# Autodesk Inventor assembly: Assembly1
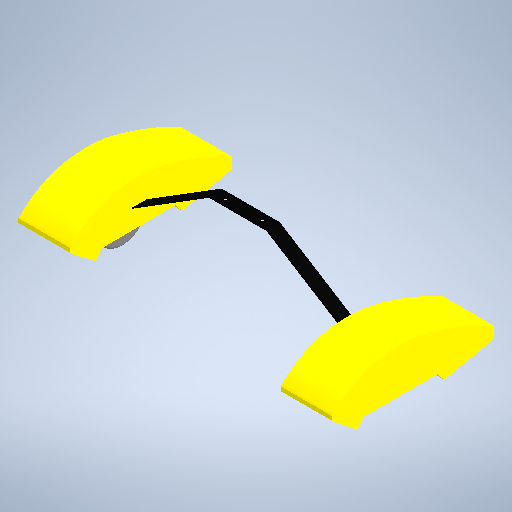
[picture p0: Inventor's stored thumbnail of the model, 512x512]
Saved by Autodesk Inventor 2025.3 (Build 293356000, 356)
## iProperties
Created: 2025-07-09
Part Number: Assembly1
Document SubType Name: Assembly
Designer: steve
Author: steve
## Documents named in this file (4)
- C:\Users\steve\OneDrive\Documentos\Avion\Main Gear\MainGear.iam
- C:\Users\steve\OneDrive\Documentos\Avion\Main Gear\F-WheelPants.ipt
- C:\Users\steve\OneDrive\Documentos\Avion\Main Gear\B-50mWheel.ipt
- C:\Users\steve\OneDrive\Documentos\Avion\Main Gear\A-MainGear.ipt
## Components (5 placed, 3 different names)
1. F-WheelPants:1 — Cylindrical:3
2. F-WheelPants:2 — Cylindrical:4
3. B-50mWheel:1 — Cylindrical:2
4. B-50mWheel:2 — Cylindrical:1
5. A-MainGear:1 — Cylindrical:1, Cylindrical:2, Cylindrical:3, Cylindrical:4
## Relationships (4: CylindricalJoint 4)
- Cylindrical:1: B-50mWheel:2 ↔ A-MainGear:1
- Cylindrical:2: B-50mWheel:1 ↔ A-MainGear:1
- Cylindrical:3: F-WheelPants:1 ↔ A-MainGear:1
- Cylindrical:4: F-WheelPants:2 ↔ A-MainGear:1
